# Autodesk Inventor assembly: ducted Fan
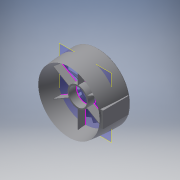
[picture p0: Inventor's stored thumbnail of the model, 180x180]
Saved by Autodesk Inventor 2018 (Build 220112000, 112)
## iProperties
Created: 2018-01-09
Part Number: ducted Fan
Document SubType Name: Assembly
Designer: mzhang
Author: mzhang
## Documents named in this file (3)
- C:\Users\mzhang\3D Objects\ducted Fan.iam
- C:\Users\mzhang\3D Objects\betterDuct.ipt
- C:\Users\mzhang\3D Objects\betterFan.ipt
## Components (2 placed, 2 different names)
1. betterDuct:1 — Mate:1
2. betterFan:1 — Mate:1
## Relationships (1: Mate 1)
- Mate:1: betterDuct:1 ↔ betterFan:1
